# Autodesk Inventor assembly: click magnet assembly
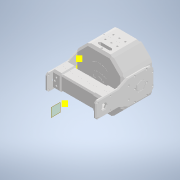
[picture p0: Inventor's stored thumbnail of the model, 180x180]
Saved by Autodesk Inventor 2022 (Build 260153000, 153)
## iProperties
Created: 2023-03-09
Part Number: click magnet assembly
Document SubType Name: Assembly
Designer: chris
Author: chris
## Documents named in this file (7)
- C:\Users\chris\Desktop\STL files\click magnet\click magnet assembly.iam
- C:\Users\chris\Desktop\STL files\click magnet\magnetbox.ipt
- C:\Users\chris\Desktop\STL files\click magnet\magnetic connector.ipt
- C:\Users\chris\Desktop\STL files\click magnet\magnet handle bracket.ipt
- C:\Users\chris\Desktop\STL files\click magnet\magnet handle bottom.ipt
- C:\Users\chris\Desktop\STL files\click magnet\magnet handle top.ipt
- C:\Users\chris\Desktop\STL files\click magnet\front brackets magnet.ipt
## Components (7 placed, 6 different names)
1. magnetbox:1 — Mate:1, Mate:2, Mate:3, Mate:12, Mate:15, Mate:17, Mate:18
2. magnetic connector:1 — Mate:4, Mate:5, Mate:13, Mate:14, Mate:16, Mate:17
3. magnet handle bracket:1 — Mate:1, Mate:2, Mate:3, Mate:4, Mate:5, Mate:6, Mate:7, Mate:8, Mate:9, Mate:10, Mate:11
4. magnet handle bottom:1 — Mate:6, Mate:7, Mate:8
5. magnet handle top:1 — Mate:9, Mate:10, Mate:11
6. magnet handle bracket:2 — Mate:12, Mate:13, Mate:14
7. front brackets magnet:1 — Mate:15, Mate:16, Mate:18
## Relationships (18: Mate 18)
- Mate:1: magnetbox:1 ↔ magnet handle bracket:1
- Mate:2: magnetbox:1 ↔ magnet handle bracket:1
- Mate:3: magnetbox:1 ↔ magnet handle bracket:1
- Mate:4: magnetic connector:1 ↔ magnet handle bracket:1
- Mate:5: magnetic connector:1 ↔ magnet handle bracket:1
- Mate:6: magnet handle bracket:1 ↔ magnet handle bottom:1
- Mate:7: magnet handle bracket:1 ↔ magnet handle bottom:1
- Mate:8: magnet handle bracket:1 ↔ magnet handle bottom:1
- Mate:9: magnet handle bracket:1 ↔ magnet handle top:1
- Mate:10: magnet handle bracket:1 ↔ magnet handle top:1
- Mate:11: magnet handle bracket:1 ↔ magnet handle top:1
- Mate:12: magnetbox:1 ↔ magnet handle bracket:2
- Mate:13: magnetic connector:1 ↔ magnet handle bracket:2
- Mate:14: magnetic connector:1 ↔ magnet handle bracket:2
- Mate:15: magnetbox:1 ↔ front brackets magnet:1
- Mate:16: magnetic connector:1 ↔ front brackets magnet:1
- Mate:17: magnetbox:1 ↔ magnetic connector:1
- Mate:18: magnetbox:1 ↔ front brackets magnet:1
